# Autodesk Inventor assembly: panelE_onFrame
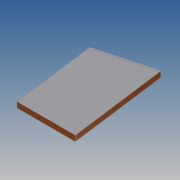
[picture p0: Inventor's stored thumbnail of the model, 180x180]
Saved by Autodesk Inventor 2014 SP1 (Build 180222100, 222)
## iProperties
Created: 2015-04-29
Part Number: panelE_onFrame
Document SubType Name: Assembly
Designer: Dave
Author: Dave
## Documents named in this file (3)
- C:\Users\Dave\Desktop\hera-cad\surface\panels\panelE_onFrame.iam
- C:\Users\Dave\Desktop\hera-cad\surface\panels\panelEframe.ipt
- C:\Users\Dave\Desktop\hera-cad\surface\panels\panelEflat.ipt
## Components (2 placed, 2 different names)
1. panelEframe:1 — Flush:1, Flush:2, Mate:1
2. panelEflat:1 — Flush:1, Flush:2, Mate:1
## Relationships (3: Flush 2, Mate 1)
- Flush:1: panelEframe:1 ↔ panelEflat:1
- Flush:2: panelEframe:1 ↔ panelEflat:1
- Mate:1: panelEframe:1 ↔ panelEflat:1
